# Autodesk Inventor assembly: ATP26MXL025-B-P6
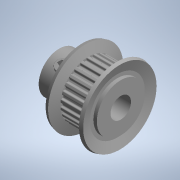
[picture p0: Inventor's stored thumbnail of the model, 180x180]
Saved by Autodesk Inventor 2022 (Build 260153000, 153)
## iProperties
Part Number: ATP26MXL025-B-P6
Catalog Web Link: www.cadenas.de
Description: ATP__MXL013, ATP__MXL019, ATP__MXL025, ATP__MXL037, ATP__MXL050, BTP__MXL013, BTP__MXL019, BTP__MXL025, BTP__MXL037, BTP__MXL050, KTP__MXL013, KTP__MXL019, KTP__MXL025, KTP__MXL037, KTP__MXL050, NTP__MXL013, NTP__MXL019, NTP__MXL025, NTP__MXL037, NTP__MXL050, MTP__MXL025, MTP__MXL037, MTPB__MXL025, MTPB__MXL037, MTPP__MXL025, MTPP__MXL037, STP__MXL025, STP__MXL037-Timing Pulleys MXL Type
Vendor: MISUMI
Document SubType Name: Assembly
Designer: partserver
Manufacturer: MISUMI
Mass: 2.74898 g
Surface Area: 25.4344 cm^2
Volume: 2.74898 cm^3
Density: 1 g/cm^3
Category: PARTsolutions
Company: MISUMI
PSOL_IDENT_0: {$CADENAS_DATA\23d-libs\misumi\metric\51_timing_pulleys\mtp_mxl_asmtab.prj},784 {VTYP=3D},{STYP=ASST
PSOL_IDENT_1: AB},{NB=ATP26MXL025-B-P6},{LINA=ATP26MXL025-B-P6},{NN=ATP__MXL013, ATP__MXL019, ATP__MXL025, ATP__MX
PSOL_IDENT_2: L037, ATP__MXL050, BTP__MXL013, BTP__MXL019, BTP__MXL025, BTP__MXL037, BTP__MXL050, KTP__MXL013, KTP
PSOL_IDENT_3: __MXL019, KTP__MXL025, KTP__MXL037, KTP__MXL050, NTP__MXL013, NTP__MXL019, NTP__MXL025, NTP__MXL037,
PSOL_IDENT_4: NTP__MXL050, MTP__MXL025, MTP__MXL037, MTPB__MXL025, MTPB__MXL037, MTPP__MXL025, MTPP__MXL037, STP_
PSOL_IDENT_5: _MXL025, STP__MXL037},{DATE=21.06.2021 00:27:39},{GEOMDATE=14.06.2021 09:50:44},{VERSION=},{LINEID=1
PSOL_IDENT_6: 30},{WBVAR=MATP,ST,TNW,PS,SBS,DD,Z,J,Q,R,S,T,ALT1,ALT2,M,QSC,QFC,QTC,ALT3,K,KSC,KFC,KTC,ALT4,ZM,ZSC,
PSOL_IDENT_7: ZFC,ZTC,ALT5,ALT6,ALT7,FC,ALT8,SRG,ALT9,BTC,TL,ALT10,TPC,ALT11,BC,ALT12,SLH},{WBNUMERIC=DD,Z,J,Q,R,S
PSOL_IDENT_8: ,T,QSC,QFC,QTC,K,KSC,KFC,KTC,ZSC,ZFC,ZTC,FC,SRG,BTC,TL,BC,SLH}  {NB=ATP26MXL025-B-P6},{LINA=ATP26MXL
PSOL_IDENT_9: 025-B-P6},{KT=DUMMY},{PN=ATP26MXL025-B-P6},{TYPE=ATP},{MATP=A2017},{MATPALG= 'A2017','Aluminum Alloy
PSOL_IDENT_10: 2000 series','S45C','1045 Carbon Steel Equivalent','SUS304','SUS304' },{ST=CA},{STALG= 'CA','Clear
PSOL_IDENT_11: Anodize','BA','Black Anodize','HAT','Hard Clear Anodize','ENP','Electroless Nickel Plating' },{NT=26
PSOL_IDENT_12: },{TNW=MXL025},{TNWALG= 'MXL013','MXL019','MXL025','MXL037','MXL050' },{BW=6.4mm (1/4inch)},{PS=B},{
PSOL_IDENT_13: PSALG= 'A','B' },{SBS=P},{SBSALG= 'H','Round Hole','P','Round Hole + Tap','V','Stepped Hole','F','St
PSOL_IDENT_14: epped Hole (Counterbore holes on the boss side)' },{DD=6.00},{DDALG=[3:4/1],4.5,[5:6/1],6.35,[7:9/1]
PSOL_IDENT_15: },{DDHA=},{DDNA=},{DDNK=[10:10/1]},{DDCA=},{DDVA=},{DDY=},{DDWB=},{DDHBK=[3:4/1],4.5,[5:6/1],6.35,[7
PSOL_IDENT_16: :8/1]},{DDPBK=[3:4/1],4.5,[5:6/1],6.35,[7:9/1]},{DDNB=},{DDCB=},{DDVFB=[3:4/1],4.5,[5:6/1]},{Z=0},{Z
PSOL_IDENT_17: ALG=[0]},{ZMIN=8.000},{ZAMAX=0.000},{ZBMAX=8.000},{DDZ=6.000},{J=0.0},{JALG=[0]},{JMIN=2.000},{JMAX=
PSOL_IDENT_18: 16.000},{JPN=},{Q=0},{QALG=[0]},{QRMIN=8.000},{QRMAX=10},{WBQMIN=10.000},{R=0},{RALG=[0]},{WBRMAX=-2
PSOL_IDENT_19: .000},{S=0.0},{SALG=[0]},{SMAX=5.5},{T=0.0},{TALG=[0]},{TMAX=7},{SBSPN=-P6},{A=7.5},{W=11.5},{L=18.0
PSOL_IDENT_20: },{PD=16.82},{OD=16.31},{D=12},{DALG=12.000},{DE=12},{F=22},{E=14},{TT=1.0},{BBK=0.000},{TTK=0.0},{A
PSOL_IDENT_21: LT1=},{ALT1ALG= '','w/o KC90 (Set Screw Angle)','KC90','with KC90 (Set Screw Angle)' },{ANG=120.000}
PSOL_IDENT_22: ,{ALT1PN=},{ALT2=},{ALT2ALG= '','Not applicable' },{M=N/A},{MALG= 'N/A' },{MFTALG= 'N/A' },{MSALG= '
PSOL_IDENT_23: N/A' },{M3D=0.000},{KDML=0.000},{ML=0.000},{MUL=0.000},{PITCH=0.000},{QSC=0.0},{QSCALG=0},{QFC=0.0},
PSOL_IDENT_24: {QFCALG=0},{QTC=0.0},{QTCALG=0},{QPCDMIN=0.000},{QPCDMINALG=0.000},{QPCDMAX=8.000},{ALT2PN=},{TAP=0.
PSOL_IDENT_25: 000},{ALT3=},{ALT3ALG= '','Not applicable' },{K=0.0},{KALG=0},{KMIN=4.000},{KFTMAX=0.000},{KSMAX=0.0
PSOL_IDENT_26: 00},{KSC=0.0},{KSCALG=0},{KFC=0.0},{KFCALG=0},{KTC=0.0},{KTCALG=0},{KSCMIN=10.000},{KPCDMIN=10.000},
PSOL_IDENT_27: {KPCDMINALG=10.000},{KPCDMAX=8.000},{ALT3PN=},{ALT4=},{ALT4ALG= '','Not applicable' },{ALT4MIN=16.50
PSOL_IDENT_28: 0},{ALT4MAX=3.500},{ZM=N/A},{ZMALG= 'N/A' },{ZMFTALG= 'N/A' },{ZMSALG= 'N/A' },{ZMDD1=0.0},{ZMDD2=0.
PSOL_IDENT_29: 0},{ZMHH=0.0},{ZSC=0.0},{ZSCALG=[0]},{ZFC=0.0},{ZFCALG=[0]},{ZTC=0.0},{ZTCALG=[0]},{ZPCDMIN=0.000},{
PSOL_IDENT_30: ZPCDMINALG=0.000},{ZPCDMAX=8.000},{ALT4PN=},{ALT5=},{ALT5ALG= '','w/o Flange not Attached','NFC','wi
PSOL_IDENT_31: th NFC (Flange not Attached)' },{ALT5PN=},{ALT6=},{ALT6ALG= '','w/o Flange Attached on One Side Only'
PSOL_IDENT_32: ,'RFC','with RFC (Flange Attached on The Boss Side Only)','LFC','with LFC (Flange Attached on The Op
PSOL_IDENT_33: posite Side Only)' },{ALT6PN=},{ALT7=},{ALT7ALG= '','w/o FC (Flange Cut)','FC','with FC (Flange Cut)'
PSOL_IDENT_34: },{FC=0.0},{FCALG=0},{FCMIN=17.5},{FCMAX=20.0},{ALT7PN=},{ALT8=},{ALT8ALG= '','Not applicable' },{A
PSOL_IDENT_35: LT8ALGALG=8.000},{ALT8DD2=0.000},{ALT8MM=0.000},{ALT8NN=0.000},{QC=0.000},{KC=0.000},{ZC=0.000},{SRG=
PSOL_IDENT_36: 0.0},{SRGALG=[0]},{SRGMAX=0.0},{SRGMAX1=0.000},{DD2=0.0},{MM=0.00},{NN=0.00},{ALT8PN=},{ALT9=},{ALT9
PSOL_IDENT_37: ALG= '','Not applicable' },{BTC9=8.000},{TL9=1.000},{BTC=0},{BTCALG=[0]},{TL=0.0},{TLALG=0},{TLMIN=1
PSOL_IDENT_38: .000},{TLMAX=-12.000},{BTCL=0.0},{BTCD=0.0},{ALT9PN=},{WLBCTL=18.000},{ALT10=},{ALT10ALG= '','w/o TP
PSOL_IDENT_39: C (Tapped Hole Dimension)','TPC','with TPC (Tapped Hole Dimension)' },{TPC=N/A},{TPCALG= 'N/A' },{TP
PSOL_IDENT_40: CM=4.000},{ALT10PN=},{ALT11=},{ALT11ALG= '','Not applicable' },{BC=0.0},{BCALG=0},{BCMIN=7},{BCMAX=6
PSOL_IDENT_41: },{M1WBC=14.5},{ALT11PN=},{KTT=3},{ALT12=},{ALT12ALG= '','w/o SLH (Set Screw Length)','SLH','with SL
PSOL_IDENT_42: H (Set Screw Length)' },{SLH=0},{SLHALG=[0]},{ALT12PN=},{AC=M4x3},{M1=4.000},{M1L=3.000},{TEDEG=20.0
PSOL_IDENT_43: 00},{TEB=0.670},{PPATH=mtp_mxl/atp_mxl_asmtpl.prj}
NB: ATP26MXL025-B-P6
NN: 0
NT: 26
NBSYN: $PN.
LINA: ATP26MXL025-B-P6
CATALOG: Misumi
PN: ATP26MXL025-B-P6
MATP: Aluminum Alloy 2000 series
ST: Clear Anodize
TNW: MXL025
BW: 6.4mm (1/4inch)
PS: B
SBS: Round Hole + Tap
DD: 6
Z: 0
J: 0
Q: 0
R: 0
S: 0
T: 0
A: 7.5
W: 11.5
L: 18
PD: 16.82
OD: 16.31
D: 12
F: 22
E: 14
ALT1: w/o KC90 (Set Screw Angle)
ALT2: Not applicable
M: N/A
QSC: 0
QFC: 0
QTC: 0
ALT3: Not applicable
K: 0
KSC: 0
KFC: 0
KTC: 0
ALT4: Not applicable
ZM: N/A
ZMDD1: 0
ZMDD2: 0
ZMHH: 0
ZSC: 0
ZFC: 0
ZTC: 0
ALT5: w/o Flange not Attached
ALT6: w/o Flange Attached on One Side Only
ALT7: w/o FC (Flange Cut)
FC: 0
ALT8: Not applicable
SRG: 0
DD2: 0
MM: 0
ALT9: Not applicable
BTC: 0
TL: 0
BTCL: 0
BTCD: 0
ALT10: w/o TPC (Tapped Hole Dimension)
TPC: N/A
ALT11: Not applicable
BC: 0
ALT12: w/o SLH (Set Screw Length)
SLH: 0
AC: M4x3
SUPPLIER: MISUMI
ARTICLENO: ATP26MXL025-B-P6
BOMINFO: ATP26MXL025-B-P6
CREATOR: CADENAS GmbH
Title: ATP26MXL025-B-P6
Author: Cadenas PARTsolutions
Comments: Timing Pulleys MXL Type
## Documents named in this file (3)
- C:\Users\yuto6\Box\Public_Share\キャチロボバトルコンテスト2021\CAD\catchrobo_hardware\assy-shooter\ATP26MXL025-B-P6.iam
- C:\Users\yuto6\Box\Public_Share\キャチロボバトルコンテスト2021\CAD\catchrobo_hardware\assy-shooter\ATP26MXL025-B-P6_b.ipt
- C:\Users\yuto6\Box\Public_Share\キャチロボバトルコンテスト2021\CAD\catchrobo_hardware\assy-shooter\SET-SCREW4-3.ipt
## Components (3 placed, 2 different names)
1. ATP26MXL025-B-P6_b:1 — to_screw1_Z@1 <-> CP_Z@2, to_screw2_Z@1 <-> CP_Z@3
2. SET-SCREW4-3:1 — to_screw1_Z@1 <-> CP_Z@2
3. SET-SCREW4-3:2 — to_screw2_Z@1 <-> CP_Z@3
## Relationships (2: Mate 2)
- to_screw1_Z@1 <-> CP_Z@2 [Mate]: ATP26MXL025-B-P6_b:1 ↔ SET-SCREW4-3:1
- to_screw2_Z@1 <-> CP_Z@3 [Mate]: ATP26MXL025-B-P6_b:1 ↔ SET-SCREW4-3:2
